# Autodesk Inventor assembly: Master
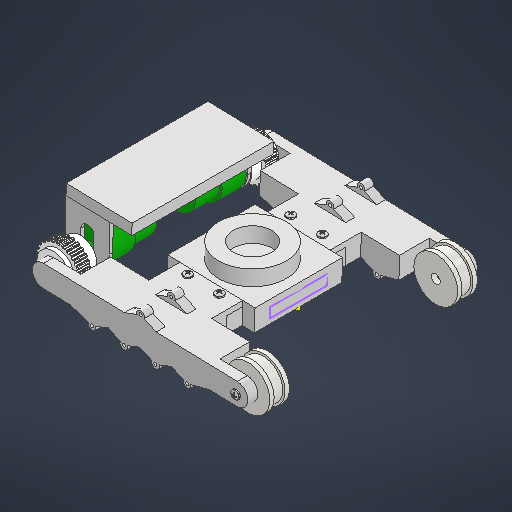
[picture p0: Inventor's stored thumbnail of the model, 512x512]
Saved by Autodesk Inventor 2026.2 (Build 302298010, 298A)
## iProperties
Created: 2026-06-22
Part Number: Master
Document SubType Name: Assembly
Designer: Inigo Greenall
Author: Inigo Greenall
## iProperties of the stored document 90592A090_Steel Hex Nut.ipt
Company: McMaster Carr Supply
Created: 2026-06-01
Part Number: 90592A090_Steel Hex Nut
Material: Generic
Description: STEP AP203
Document SubType Name: Modeling
Designer: Inigo Greenall
Density: 1 g/cm^3
Appearance: Default
Mass: 0.101732 g
Surface Area: 1.92468 cm^2
Volume: 0.101732 cm^3
Sending System: SolidWorks 2024
Preprocessor: SwSTEP 2.0
Title: 90592A090_Steel Hex Nut.STEP
Author: McMaster Carr Supply
Revision Number: ANY
## iProperties of the stored document 92000A230_Passivated 18-8 Stainless Steel Pan Head Phillips Screws.ipt
Company: McMaster Carr Supply
Created: 2026-01-08
Part Number: 92000A230_Passivated 18-8 Stainless Steel Pan Head Phillips Screws
Material: Generic
Description: STEP AP203
Document SubType Name: Modeling
Designer: Inigo Greenall
Density: 1 g/cm^3
Appearance: Default
Mass: 0.364738 g
Surface Area: 6.2915 cm^2
Volume: 0.364738 cm^3
Sending System: SolidWorks 2024
Preprocessor: SwSTEP 2.0
Title: 92000A230_Passivated 18-8 Stainless Steel Pan Head Phillips Screws.STEP
Author: McMaster Carr Supply
Revision Number: ANY
## Documents named in this file (12)
- C:\Users\Inigo Greenall\OneDrive\excavator-project\hardware\Master.iam
- C:\Users\Inigo Greenall\OneDrive\excavator-project\hardware\Motor\Motor Stand Assembly.iam
- C:\Users\Inigo Greenall\OneDrive\excavator-project\hardware\synchronous-belt\Synchronous Belts Transmission2.iam
- C:\Users\Inigo Greenall\OneDrive\excavator-project\hardware\Base\Base Plate.iam
- C:\Users\Inigo Greenall\OneDrive\excavator-project\hardware\Bearing.ipt
- **C:\Users\Inigo Greenall\OneDrive\excavator-project\hardware\Master.iam*LocalDocs*xAaaaqpaaAaaaaaaaAaaaqmrzIc*92000A230_Passivated 18-8 Stainless Steel Pan Head Phillips Screws.ipt
- **C:\Users\Inigo Greenall\OneDrive\excavator-project\hardware\Master.iam*LocalDocs*xAaaaqkbaAaaaaaaaAaaaaj1j2a*90592A090_Steel Hex Nut.ipt
- C:\Users\Inigo Greenall\OneDrive\excavator-project\hardware\Bridge Plate.ipt
- **C:\Users\icgre\OneDrive\Excavator Project\Master.iam*LocalDocs*xAaaaqkbaAaaaaaaaAaaaaj1j2a*90592A090_Steel Hex Nut.ipt
- **C:\Users\icgre\OneDrive\Excavator Project\Master.iam*LocalDocs*xAaaaqpaaAaaaaaaaAaaaqmrzIc*92000A230_Passivated 18-8 Stainless Steel Pan Head Phillips Screws.ipt
- C:\Users\Inigo Greenall\OneDrive\excavator-project\hardware\92000A230_Passivated 18-8 Stainless Steel Pan Head Phillips Screws.STEP
- C:\Users\Inigo Greenall\OneDrive\excavator-project\hardware\90592A090_Steel Hex Nut.STEP
## Components (19 placed, 7 different names)
1. Motor Stand Assembly:1 [sub-assembly] — Mate:8, Mate:11, Angle:1, Flush:1, Mate:20, Flush:2
2. Motor Stand Assembly:2 [sub-assembly] — Mate:9, Mate:10, Angle:1, Angle:2
3. Synchronous Belts Transmission:1 [sub-assembly] — Mate:6, Mate:7, Mate:8, Mate:11, Angle:2, Mate:19, Insert:14
4. Synchronous Belts Transmission:2 [sub-assembly] — Mate:6, Mate:7, Mate:9, Mate:10, Mate:16, Mate:17, Mate:18, Insert:16
5. Base Plate:1 [sub-assembly] — Mate:16, Mate:17, Mate:18, Mate:19, Insert:5, Insert:6, Insert:7, Insert:8, Insert:9, Insert:10, Insert:11, Insert:12, Insert:13, Insert:15
6. Bearing:1
7. Bridge Plate:1 — Flush:1, Mate:20, Flush:2
8. 90592A090_Steel Hex Nut:6 — Insert:16
9. 90592A090_Steel Hex Nut:1 — Insert:10
10. 90592A090_Steel Hex Nut:2 — Insert:11
11. 90592A090_Steel Hex Nut:3 — Insert:12
12. 90592A090_Steel Hex Nut:4 — Insert:13
13. 90592A090_Steel Hex Nut:5 — Insert:14
14. 92000A230_Passivated 18-8 Stainless Steel Pan Head Phillips Screws:6 — Insert:15
15. 92000A230_Passivated 18-8 Stainless Steel Pan Head Phillips Screws:2 — Insert:9
16. 92000A230_Passivated 18-8 Stainless Steel Pan Head Phillips Screws:3 — Insert:6
17. 92000A230_Passivated 18-8 Stainless Steel Pan Head Phillips Screws:4 — Insert:7
18. 92000A230_Passivated 18-8 Stainless Steel Pan Head Phillips Screws:5 — Insert:8
19. 92000A230_Passivated 18-8 Stainless Steel Pan Head Phillips Screws:1 — Insert:5
## Relationships (27: Insert 12, Mate 11, Angle 2, Flush 2)
- Mate:6: Synchronous Belts Transmission:1 ↔ Synchronous Belts Transmission:2
- Mate:7: Synchronous Belts Transmission:1 ↔ Synchronous Belts Transmission:2
- Mate:8: Motor Stand Assembly:1 ↔ Synchronous Belts Transmission:1
- Mate:9: Motor Stand Assembly:2 ↔ Synchronous Belts Transmission:2
- Mate:10: Motor Stand Assembly:2 ↔ Synchronous Belts Transmission:2
- Mate:11: Motor Stand Assembly:1 ↔ Synchronous Belts Transmission:1
- Angle:1 (0 deg): Motor Stand Assembly:1 ↔ Motor Stand Assembly:2
- Angle:2 (0 deg): Motor Stand Assembly:2 ↔ Synchronous Belts Transmission:1
- Mate:16: Synchronous Belts Transmission:2 ↔ Base Plate:1
- Mate:17: Synchronous Belts Transmission:2 ↔ Base Plate:1
- Mate:18: Synchronous Belts Transmission:2 ↔ Base Plate:1
- Mate:19: Synchronous Belts Transmission:1 ↔ Base Plate:1
- Insert:5: Base Plate:1 ↔ 92000A230_Passivated 18-8 Stainless Steel Pan Head Phillips Screws:1
- Insert:6: Base Plate:1 ↔ 92000A230_Passivated 18-8 Stainless Steel Pan Head Phillips Screws:3
- Insert:7: Base Plate:1 ↔ 92000A230_Passivated 18-8 Stainless Steel Pan Head Phillips Screws:4
- Insert:8: Base Plate:1 ↔ 92000A230_Passivated 18-8 Stainless Steel Pan Head Phillips Screws:5
- Insert:9: Base Plate:1 ↔ 92000A230_Passivated 18-8 Stainless Steel Pan Head Phillips Screws:2
- Insert:10: Base Plate:1 ↔ 90592A090_Steel Hex Nut:1
- Insert:11: Base Plate:1 ↔ 90592A090_Steel Hex Nut:2
- Insert:12: Base Plate:1 ↔ 90592A090_Steel Hex Nut:3
- Insert:13: Base Plate:1 ↔ 90592A090_Steel Hex Nut:4
- Insert:14: Synchronous Belts Transmission:1 ↔ 90592A090_Steel Hex Nut:5
- Insert:15: Base Plate:1 ↔ 92000A230_Passivated 18-8 Stainless Steel Pan Head Phillips Screws:6
- Flush:1: Motor Stand Assembly:1 ↔ Bridge Plate:1
- Mate:20: Motor Stand Assembly:1 ↔ Bridge Plate:1
- Flush:2: Motor Stand Assembly:1 ↔ Bridge Plate:1
- Insert:16: Synchronous Belts Transmission:2 ↔ 90592A090_Steel Hex Nut:6
